# Autodesk Inventor assembly: 200-50-WHEEL-CONNECTOR-ASM-01
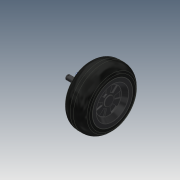
[picture p0: Inventor's stored thumbnail of the model, 180x180]
Saved by Autodesk Inventor 2018.2 (Build 222227000, 227)
## iProperties
Created: 2017-12-17
Part Number: 200-50-WHEEL-CONNECTOR-ASM-01
Document SubType Name: Assembly
Designer: feesmrt
Author: feesmrt
## Documents named in this file (3)
- D:\Programmierung\FRANC0R\CAD\02-Rocker-Bogie-Robot\200-ROCKER-BOGIE\200-50-WHEEL-CONNECTOR\200-50-WHEEL-CONNECTOR-ASM-01.iam
- D:\Programmierung\FRANC0R\CAD\02-Rocker-Bogie-Robot\200-ROCKER-BOGIE\200-50-WHEEL-CONNECTOR\200-50-WHEEL-CONNECTOR-01.ipt
- D:\Programmierung\FRANC0R\CAD\02-Rocker-Bogie-Robot\900-COMPONENTS\900-10-WHEEL\900-10-WHEEL-ASM-01.iam
## Components (2 placed, 2 different names)
1. 200-50-WHEEL-CONNECTOR-01:1 — Fluchtend:2, Fluchtend:1, Passend:1
2. 900-10-WHEEL-ASM-01:1 [sub-assembly] — Fluchtend:2, Fluchtend:1, Passend:1
## Relationships (3: Flush 2, Mate 1)
- Fluchtend:2 [Flush]: 200-50-WHEEL-CONNECTOR-01:1 ↔ 900-10-WHEEL-ASM-01:1
- Fluchtend:1 [Flush] (18.5 mm): 200-50-WHEEL-CONNECTOR-01:1 ↔ 900-10-WHEEL-ASM-01:1
- Passend:1 [Mate] (5 mm): 200-50-WHEEL-CONNECTOR-01:1 ↔ 900-10-WHEEL-ASM-01:1
